# Autodesk Inventor assembly: Förderband
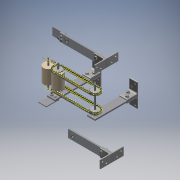
[picture p0: Inventor's stored thumbnail of the model, 180x180]
Saved by Autodesk Inventor 2018 (Build 220112000, 112)
## iProperties
Created: 2018-01-11
Part Number: Förderband
Material: Generisch
Document SubType Name: Assembly
Designer: Dominik
Author: Dominik
## Documents named in this file (10)
- C:\Users\Julian\Desktop\Schule\5AHME\Diplomarbeit\Git\fuettr_prototype\Mechanical\Inventorskizzen\Förderband.iam
- C:\Users\Julian\Desktop\Schule\5AHME\Diplomarbeit\Git\fuettr_prototype\Mechanical\Inventorskizzen\Kettenradzusammensetzung_links.iam
- C:\Users\Julian\Desktop\Schule\5AHME\Diplomarbeit\Git\fuettr_prototype\Mechanical\Inventorskizzen\Förderbandwelle_vorne.ipt
- C:\Users\Julian\Desktop\Schule\5AHME\Diplomarbeit\Git\fuettr_prototype\Mechanical\Inventorskizzen\Förderbandwelle_hinten.ipt
- C:\Users\Julian\Desktop\Schule\5AHME\Diplomarbeit\Git\fuettr_prototype\Mechanical\Inventorskizzen\Kunststoffrolle_antrieb.ipt
- C:\Users\Julian\Desktop\Schule\5AHME\Diplomarbeit\Git\fuettr_prototype\Mechanical\Inventorskizzen\Auspressrolle_befaesstigung.iam
- C:\Users\Julian\Documents\Inventor\Content Center Files\R2018\de-DE\DIN 471(1)\DIN 471 - 8x0,8.ipt
- C:\Users\Julian\Documents\Inventor\Content Center Files\R2018\de-DE\IS 2048  A\IS 2048 - 1983 - Spezifikation für Passfedern und Keilnute A 3 x 3 x 6.ipt
- C:\Users\Julian\Desktop\Schule\5AHME\Diplomarbeit\Git\fuettr_prototype\Mechanical\Inventorskizzen\Lagerhalterung.iam
- C:\Users\Julian\Desktop\Schule\5AHME\Diplomarbeit\Git\fuettr_prototype\Mechanical\Inventorskizzen\Lagerhalterung_ohne_Platte.iam
## Components (26 placed, 9 different names)
1. Kettenradzusammensetzung_links:1 [sub-assembly] — Starr:2, Starr:5, Starr:6, Starr:15
2. Kettenradzusammensetzung_links:2 [sub-assembly] — Starr:1, Starr:4, Starr:13
3. Kunststoffrolle_antrieb:1 — Starr:3, Passend:1
4. Förderbandwelle_hinten:1 — Starr:4, Starr:5, Starr:7, Starr:8, Starr:9, Starr:10, Starr:17
5. Förderbandwelle_vorne:1 — Starr:1, Starr:2, Starr:3, Drehbar:1, Starr:11, Starr:12, Starr:14, Starr:16, Zylindrisch:1, Starr:18
6. Auspressrolle_befaesstigung:1 [sub-assembly] — Zylindrisch:1, Passend:1
7. DIN 471 8x0,8:1 — Starr:7
8. DIN 471 8x0,8:2 — Starr:6
9. DIN 471 8x0,8:3 — Starr:13
10. DIN 471 8x0,8:4
11. DIN 471 8x0,8:5 — Starr:16
12. DIN 471 8x0,8:8
13. DIN 471 8x0,8:6
14. DIN 471 8x0,8:7 — Starr:15
15. DIN 471 8x0,8:9 — Starr:14
16. DIN 471 8x0,8:10
17. DIN 471 8x0,8:11 — Starr:12
18. DIN 471 8x0,8:12 — Starr:8
19. IS 2048 A Spezifikation für Passfedern und Keilnute A 3 x 3 x 6:1 — Drehbar:1
20. IS 2048 A Spezifikation für Passfedern und Keilnute A 3 x 3 x 6:2 — Starr:10
21. IS 2048 A Spezifikation für Passfedern und Keilnute A 3 x 3 x 6:3 — Starr:9
22. IS 2048 A Spezifikation für Passfedern und Keilnute A 3 x 3 x 6:4 — Starr:11
23. Lagerhalterung:1 [sub-assembly]
24. Lagerhalterung:2 [sub-assembly] — Starr:18
25. Lagerhalterung_ohne_Platte:1 [sub-assembly]
26. Lagerhalterung_ohne_Platte:2 [sub-assembly] — Starr:17
## Relationships (21: WeldJoint 18, RevoluteJoint 1, CylindricalJoint 1, Mate 1)
- Starr:1 [WeldJoint]: Kettenradzusammensetzung_links:2 ↔ Förderbandwelle_vorne:1
- Starr:2 [WeldJoint]: Kettenradzusammensetzung_links:1 ↔ Förderbandwelle_vorne:1
- Starr:3 [WeldJoint]: Kunststoffrolle_antrieb:1 ↔ Förderbandwelle_vorne:1
- Starr:4 [WeldJoint]: Kettenradzusammensetzung_links:2 ↔ Förderbandwelle_hinten:1
- Starr:5 [WeldJoint]: Kettenradzusammensetzung_links:1 ↔ Förderbandwelle_hinten:1
- Starr:6 [WeldJoint]: Kettenradzusammensetzung_links:1 ↔ DIN 471 8x0,8:2
- Starr:7 [WeldJoint]: Förderbandwelle_hinten:1 ↔ DIN 471 8x0,8:1
- Starr:8 [WeldJoint]: Förderbandwelle_hinten:1 ↔ DIN 471 8x0,8:12
- Starr:9 [WeldJoint]: Förderbandwelle_hinten:1 ↔ IS 2048 A Spezifikation für Passfedern und Keilnute A 3 x 3 x 6:3
- Starr:10 [WeldJoint]: Förderbandwelle_hinten:1 ↔ IS 2048 A Spezifikation für Passfedern und Keilnute A 3 x 3 x 6:2
- Drehbar:1 [RevoluteJoint]: Förderbandwelle_vorne:1 ↔ IS 2048 A Spezifikation für Passfedern und Keilnute A 3 x 3 x 6:1
- Starr:11 [WeldJoint]: Förderbandwelle_vorne:1 ↔ IS 2048 A Spezifikation für Passfedern und Keilnute A 3 x 3 x 6:4
- Starr:12 [WeldJoint]: Förderbandwelle_vorne:1 ↔ DIN 471 8x0,8:11
- Starr:13 [WeldJoint]: Kettenradzusammensetzung_links:2 ↔ DIN 471 8x0,8:3
- Starr:14 [WeldJoint]: Förderbandwelle_vorne:1 ↔ DIN 471 8x0,8:9
- Starr:15 [WeldJoint]: Kettenradzusammensetzung_links:1 ↔ DIN 471 8x0,8:7
- Starr:16 [WeldJoint]: Förderbandwelle_vorne:1 ↔ DIN 471 8x0,8:5
- Zylindrisch:1 [CylindricalJoint]: Förderbandwelle_vorne:1 ↔ Auspressrolle_befaesstigung:1
- Passend:1 [Mate]: Kunststoffrolle_antrieb:1 ↔ Auspressrolle_befaesstigung:1
- Starr:17 [WeldJoint]: Förderbandwelle_hinten:1 ↔ Lagerhalterung_ohne_Platte:2
- Starr:18 [WeldJoint]: Förderbandwelle_vorne:1 ↔ Lagerhalterung:2
